# Autodesk Inventor assembly: Right Rear Wheel with hub shaft and pulley
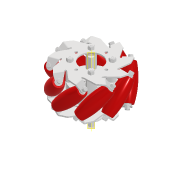
[picture p0: Inventor's stored thumbnail of the model, 180x180]
Saved by Autodesk Inventor 2020 (Build 240168000, 168)
## iProperties
Created: 2020-02-22
Part Number: Right Rear Wheel with hub shaft and pulley
Document SubType Name: Assembly
Designer: ball
Author: ball
## Documents named in this file (4)
- C:\FTC\FTC8863CAD\2019 Robot\Mecanum Drive Train Metal\Right Rear Wheel with hub shaft and pulley.iam
- C:\FTC\FTC8863CAD\2019 Robot\Mecanum Drive Train Metal\Right Rear Wheel with hub.iam
- C:\FTC\FTC8863CAD\GoBilda\2102 Parts\2102-0008-0090.ipt
- C:\FTC\FTC8863CAD\GoBilda\3414 Parts\3414-4008-0016 assembly.iam
## Components (3 placed, 3 different names)
1. Right Rear Wheel with hub:1 [sub-assembly] — Flush:1, Mate:1, Mate:2, Mate:4
2. 2102-0008-0090:1 — Flush:1, Mate:1, Mate:2, Mate:3, Mate:5
3. 3414-4008-0016 assembly:1 [sub-assembly] — Mate:3, Mate:4, Mate:5
## Relationships (6: Mate 5, Flush 1)
- Flush:1 (-25.4 mm): Right Rear Wheel with hub:1 ↔ 2102-0008-0090:1
- Mate:1: Right Rear Wheel with hub:1 ↔ 2102-0008-0090:1
- Mate:2: Right Rear Wheel with hub:1 ↔ 2102-0008-0090:1
- Mate:3: 2102-0008-0090:1 ↔ 3414-4008-0016 assembly:1
- Mate:4: Right Rear Wheel with hub:1 ↔ 3414-4008-0016 assembly:1
- Mate:5: 2102-0008-0090:1 ↔ 3414-4008-0016 assembly:1
